# Autodesk Inventor assembly: Tetrix_736468
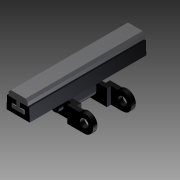
[picture p0: Inventor's stored thumbnail of the model, 180x180]
Saved by Autodesk Inventor 2015 SP1 (Build 190203100, 203)
## iProperties
Category: Add-on Components
Company: Autodesk Inc.
Created: 2014-11-23
Part Number: Tetrix_736468
Document SubType Name: Assembly
Designer: Tetrix
Catalog Web Link: http://www.tetrixrobotics.com/TETRIX_Tank_Tread_Kit
Vendor: Tetrix
Author: Autodesk Inc.
## Documents named in this file (3)
- D:\Data Folder\FTC 2015\KOP\Tetrix\Tetrix_736468.iam
- D:\Data Folder\FTC 2015\KOP\Tetrix\Tetrix_736468_Link.ipt
- D:\Data Folder\FTC 2015\KOP\Tetrix\Tetrix_736468_Insert.ipt
## Components (2 placed, 2 different names)
1. Tetrix_736468_Link:1 — Flush:1, Mate:1, Mate:3, Angle:2
2. Tetrix_736468_Insert:1 — Flush:1, Mate:1, Mate:2, Angle:1
## Relationships (7: Mate 4, Angle 2, Flush 1)
- Flush:1: Tetrix_736468_Link:1 ↔ Tetrix_736468_Insert:1
- Mate:1: Tetrix_736468_Link:1 ↔ Tetrix_736468_Insert:1
- Mate:2: Tetrix_736468_Insert:1
- Angle:1 (0 deg): Tetrix_736468_Insert:1
- Mate:3: Tetrix_736468_Link:1
- Angle:2 (0 deg): Tetrix_736468_Link:1
- Mate:4
